# Autodesk Inventor assembly: 527458 SDE5-V1-O-Q6-P-M8
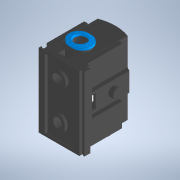
[picture p0: Inventor's stored thumbnail of the model, 180x180]
Saved by Autodesk Inventor 2021 (Build 250183000, 183)
## iProperties
Category: PARTsolutions
Company: FESTO
Created: 2026-04-21
Part Number: 527458 SDE5-V1-O-Q6-P-M8
Catalog Web Link: www.3dfindit.com
Description: SDE5-pressure sensor
Vendor: FESTO
Document SubType Name: Assembly
Designer: psAdmin
Manufacturer: FESTO
Mass: 19 g
Surface Area: 107.653 cm^2
Volume: 20.9431 cm^3
Density: 0.907221 g/cm^3
Title: 527458 SDE5-V1-O-Q6-P-M8
Author: Cadenas PARTsolutions
Comments: pressure sensor
PSOL_IDENT_0: {ATYP=ASSISTANT},{DATA=script=$CADENAS_DATA/23d-libs/festo/webfesto.vbb&M_FAMILY=SDE5&M_GROUP=01&M_P
PSOL_IDENT_1: ARTNO=527458&IDCODE1=SDE5-V1-O-Q6-P-M8&IDCODE2=&customer_number_cns=&MATES=1&LOD=HI&LOCKERP=0&SINGLE
PSOL_IDENT_2: PART=1}
NB: 527458 SDE5-V1-O-Q6-P-M8
NN: SDE5
NT: pressure sensor
NBSYN: $TNR. $TYP.
LINA: 527458 SDE5-V1-O-Q6-P-M8
CATALOG: Festo
TNR: 527458
TYP: SDE5-V1-O-Q6-P-M8
CNSMASSEXACT: 0.019
GTIN: 4052568162559
SUPPLIER: FESTO
ARTICLENO: 527458 SDE5-V1-O-Q6-P-M8
BOMINFO: 527458 SDE5-V1-O-Q6-P-M8
CREATOR: CADENAS GmbH
## Documents named in this file (3)
- e:\temp\worker_COMMON_292\temp\tmp_5448_28_11gTP\format_0\527458 SDE5-V1-O-Q6-P-M8.iam
- e:\temp\worker_COMMON_292\temp\tmp_5448_28_11gTP\format_0\527458 SDE5-Q6-M8(O)---(DS).ipt
- e:\temp\worker_COMMON_292\temp\tmp_5448_28_11gTP\format_0\653056 SDE5---(H).ipt
## Components (2 placed, 2 different names)
1. 527458 SDE5-Q6-M8(O)---(DS):1 — CLIP_XY@1 <-> ANBAU_XY@2, CLIP_Z@1 <-> ANBAU_Z@2, CLIP_YZ@1 <-> ANBAU_YZ@2
2. 653056 SDE5---(H):1 — CLIP_XY@1 <-> ANBAU_XY@2, CLIP_Z@1 <-> ANBAU_Z@2, CLIP_YZ@1 <-> ANBAU_YZ@2
## Relationships (3: Flush 1, Mate 1, Angle 1)
- CLIP_XY@1 <-> ANBAU_XY@2 [Flush]: 527458 SDE5-Q6-M8(O)---(DS):1 ↔ 653056 SDE5---(H):1
- CLIP_Z@1 <-> ANBAU_Z@2 [Mate]: 527458 SDE5-Q6-M8(O)---(DS):1 ↔ 653056 SDE5---(H):1
- CLIP_YZ@1 <-> ANBAU_YZ@2 [Angle] (0 deg): 527458 SDE5-Q6-M8(O)---(DS):1 ↔ 653056 SDE5---(H):1
